# Autodesk Inventor assembly: 組合3-2
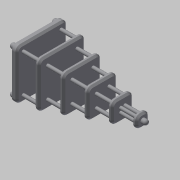
[picture p0: Inventor's stored thumbnail of the model, 180x180]
Saved by Autodesk Inventor 2018 (Build 220112000, 112)
## iProperties
Created: 2020-09-21
Part Number: 組合3-2
Material: 一般
Document SubType Name: Assembly
Designer: 王鼎鈞
Author: 王鼎鈞
## Documents named in this file (9)
- D:\2020嚴家明 功課黨\組合3-2.iam
- D:\2020嚴家明 功課黨\exercise3-1-1.ipt
- D:\2020嚴家明 功課黨\exercise3-1-2.ipt
- D:\2020嚴家明 功課黨\exercise3-1-3.ipt
- D:\2020嚴家明 功課黨\exercise3-1-4.ipt
- D:\2020嚴家明 功課黨\exercise3-1-5.ipt
- D:\2020嚴家明 功課黨\exercise3-1-6.ipt
- D:\2020嚴家明 功課黨\exercise2-6.ipt
- D:\2020嚴家明 功課黨\exercise2-7.ipt
## Components (31 placed, 8 different names)
1. exercise3-1-1:1 — 插入:1, 插入:2, 插入:3, 插入:4, 插入:6, 插入:7, 插入:8, 插入:9
2. exercise3-1-2:1 — 插入:5, 貼合:1, 插入:10, 插入:11, 插入:12, 插入:13
3. exercise3-1-3:1 — 插入:14, 插入:15, 插入:16, 插入:17, 插入:18, 插入:19
4. exercise3-1-4:1 — 插入:20, 插入:21, 插入:22, 插入:23, 插入:24, 插入:25
5. exercise3-1-5:1 — 插入:26, 插入:27, 插入:28, 插入:29, 插入:30, 插入:31
6. exercise3-1-6:1 — 插入:32, 插入:33, 插入:34
7. exercise2-6:1 — 插入:28, 插入:32
8. exercise2-6:2 — 插入:29
9. exercise2-6:3 — 插入:30
10. exercise2-6:4 — 插入:31, 插入:33
11. exercise2-6:5 — 插入:25, 插入:27
12. exercise2-6:6 — 插入:24
13. exercise2-6:7 — 插入:23
14. exercise2-6:8 — 插入:18
15. exercise2-6:9 — 插入:19, 插入:21
16. exercise2-6:10 — 插入:22, 插入:26
17. exercise2-6:11 — 插入:1, 插入:5
18. exercise2-6:12 — 插入:2
19. exercise2-6:13 — 插入:3, 貼合:1
20. exercise2-6:14 — 插入:16, 插入:20
21. exercise2-6:15 — 插入:17
22. exercise2-6:16 — 插入:13, 插入:15
23. exercise2-6:17 — 插入:12
24. exercise2-6:18 — 插入:11
25. exercise2-6:19 — 插入:10, 插入:14
26. exercise2-6:20 — 插入:4
27. exercise2-7:1 — 插入:6
28. exercise2-7:2 — 插入:7
29. exercise2-7:3 — 插入:9
30. exercise2-7:4 — 插入:8
31. exercise2-7:5 — 插入:34
## Relationships (35: Insert 34, Mate 1)
- 插入:1 [Insert]: exercise3-1-1:1 ↔ exercise2-6:11
- 插入:2 [Insert]: exercise3-1-1:1 ↔ exercise2-6:12
- 插入:3 [Insert]: exercise3-1-1:1 ↔ exercise2-6:13
- 插入:4 [Insert]: exercise3-1-1:1 ↔ exercise2-6:20
- 插入:5 [Insert]: exercise3-1-2:1 ↔ exercise2-6:11
- 貼合:1 [Mate]: exercise3-1-2:1 ↔ exercise2-6:13
- 插入:6 [Insert]: exercise3-1-1:1 ↔ exercise2-7:1
- 插入:7 [Insert]: exercise3-1-1:1 ↔ exercise2-7:2
- 插入:8 [Insert]: exercise3-1-1:1 ↔ exercise2-7:4
- 插入:9 [Insert]: exercise3-1-1:1 ↔ exercise2-7:3
- 插入:10 [Insert]: exercise3-1-2:1 ↔ exercise2-6:19
- 插入:11 [Insert]: exercise3-1-2:1 ↔ exercise2-6:18
- 插入:12 [Insert]: exercise3-1-2:1 ↔ exercise2-6:17
- 插入:13 [Insert]: exercise3-1-2:1 ↔ exercise2-6:16
- 插入:14 [Insert]: exercise3-1-3:1 ↔ exercise2-6:19
- 插入:15 [Insert]: exercise3-1-3:1 ↔ exercise2-6:16
- 插入:16 [Insert]: exercise3-1-3:1 ↔ exercise2-6:14
- 插入:17 [Insert]: exercise3-1-3:1 ↔ exercise2-6:15
- 插入:18 [Insert]: exercise3-1-3:1 ↔ exercise2-6:8
- 插入:19 [Insert]: exercise3-1-3:1 ↔ exercise2-6:9
- 插入:20 [Insert]: exercise3-1-4:1 ↔ exercise2-6:14
- 插入:21 [Insert]: exercise3-1-4:1 ↔ exercise2-6:9
- 插入:22 [Insert]: exercise3-1-4:1 ↔ exercise2-6:10
- 插入:23 [Insert]: exercise3-1-4:1 ↔ exercise2-6:7
- 插入:24 [Insert]: exercise3-1-4:1 ↔ exercise2-6:6
- 插入:25 [Insert]: exercise3-1-4:1 ↔ exercise2-6:5
- 插入:26 [Insert]: exercise3-1-5:1 ↔ exercise2-6:10
- 插入:27 [Insert]: exercise3-1-5:1 ↔ exercise2-6:5
- 插入:28 [Insert]: exercise3-1-5:1 ↔ exercise2-6:1
- 插入:29 [Insert]: exercise3-1-5:1 ↔ exercise2-6:2
- 插入:30 [Insert]: exercise3-1-5:1 ↔ exercise2-6:3
- 插入:31 [Insert]: exercise3-1-5:1 ↔ exercise2-6:4
- 插入:32 [Insert]: exercise3-1-6:1 ↔ exercise2-6:1
- 插入:33 [Insert]: exercise3-1-6:1 ↔ exercise2-6:4
- 插入:34 [Insert]: exercise3-1-6:1 ↔ exercise2-7:5
